# Autodesk Inventor assembly: WHEEL_BASE
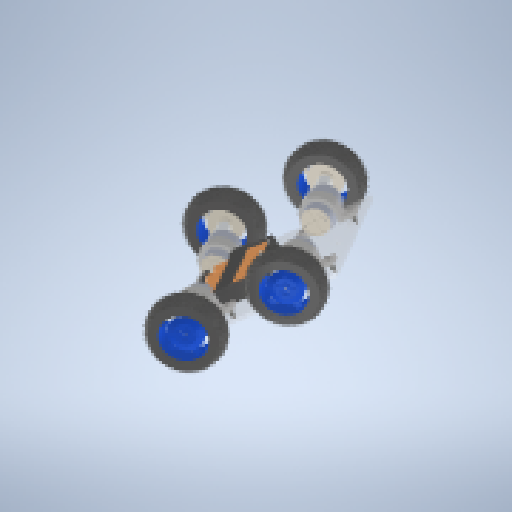
[picture p0: Inventor's stored thumbnail of the model, 512x512]
Saved by Autodesk Inventor 2025.3 (Build 293356030, 356C)
## iProperties
Created: 2026-06-30
Part Number: WHEEL_BASE
Document SubType Name: Assembly
Designer: user
Author: user
## Documents named in this file (6)
- C:\Docs\shcool\dojo\Design_3\Smaller\WHEEL_BASE.iam
- C:\Docs\shcool\dojo\Design_3\Smaller\base_2.ipt
- C:\Docs\shcool\dojo\Design_3\Smaller\motor_wheel_3.iam
- C:\Docs\shcool\dojo\Design_3\battery_case\Battery_Housing_Full.iam
- C:\Users\user\OneDrive\Documents\Inventor\Content Center Files\R2025\en-US\ISO 7040\DIEN EN ISO 7040 - M3.ipt
- C:\Users\user\OneDrive\Documents\Inventor\Content Center Files\R2025\en-US\ISO 4762(2)\ISO 4762 - M3 x 16ISO.ipt
## Components (22 placed, 5 different names)
1. base_2:1 — Mate:2, Mate:4, Mate:5, Mate:6, Mate:8, Mate:9, Mate:10, Mate:11, Mate:14, Mate:15, Mate:16, Mate:17, Mate:18, Insert:9, Insert:11, Insert:12, Insert:13, Insert:14, Insert:15, Insert:16, Insert:17
2. motor_wheel_3:1 [sub-assembly] — Mate:2, Mate:15, Mate:16, Insert:5, Insert:6
3. motor_wheel_3:2 [sub-assembly] — Mate:4, Mate:5, Mate:11, Insert:7, Insert:8
4. motor_wheel_3:3 [sub-assembly] — Mate:6, Mate:17, Mate:18, Insert:1, Insert:2
5. motor_wheel_3:4 [sub-assembly] — Mate:8, Mate:9, Mate:10, Mate:19, Insert:3, Insert:4
6. Battery_Housing_Full:1 [sub-assembly] — Mate:14, Mate:19
7. ISO 4762 M3 x 16:1 — Insert:5
8. ISO 4762 M3 x 16:2 — Insert:2
9. ISO 4762 M3 x 16:3 — Insert:3
10. ISO 4762 M3 x 16:4 — Insert:4
11. ISO 4762 M3 x 16:5 — Insert:6
12. ISO 4762 M3 x 16:6 — Insert:1
13. ISO 4762 M3 x 16:7 — Insert:7
14. ISO 4762 M3 x 16:8 — Insert:8
15. DIN EN ISO 7040 M3:3 — Insert:11
16. DIN EN ISO 7040 M3:4 — Insert:15
17. DIN EN ISO 7040 M3:5 — Insert:12
18. DIN EN ISO 7040 M3:6 — Insert:14
19. DIN EN ISO 7040 M3:7 — Insert:13
20. DIN EN ISO 7040 M3:8 — Insert:9
21. DIN EN ISO 7040 M3:9 — Insert:16
22. DIN EN ISO 7040 M3:10 — Insert:17
## Relationships (30: Insert 16, Mate 14)
- Mate:2: base_2:1 ↔ motor_wheel_3:1
- Mate:4: base_2:1 ↔ motor_wheel_3:2
- Mate:5: base_2:1 ↔ motor_wheel_3:2
- Mate:6: base_2:1 ↔ motor_wheel_3:3
- Mate:8: base_2:1 ↔ motor_wheel_3:4
- Mate:9: base_2:1 ↔ motor_wheel_3:4
- Mate:10: base_2:1 ↔ motor_wheel_3:4
- Mate:11: base_2:1 ↔ motor_wheel_3:2
- Mate:14: base_2:1 ↔ Battery_Housing_Full:1
- Mate:15: base_2:1 ↔ motor_wheel_3:1
- Mate:16: base_2:1 ↔ motor_wheel_3:1
- Mate:17: base_2:1 ↔ motor_wheel_3:3
- Mate:18: base_2:1 ↔ motor_wheel_3:3
- Mate:19 (3 mm): motor_wheel_3:4 ↔ Battery_Housing_Full:1
- Insert:1: motor_wheel_3:3 ↔ ISO 4762 M3 x 16:6
- Insert:2: motor_wheel_3:3 ↔ ISO 4762 M3 x 16:2
- Insert:3: motor_wheel_3:4 ↔ ISO 4762 M3 x 16:3
- Insert:4: motor_wheel_3:4 ↔ ISO 4762 M3 x 16:4
- Insert:5: motor_wheel_3:1 ↔ ISO 4762 M3 x 16:1
- Insert:6: motor_wheel_3:1 ↔ ISO 4762 M3 x 16:5
- Insert:7: motor_wheel_3:2 ↔ ISO 4762 M3 x 16:7
- Insert:8: motor_wheel_3:2 ↔ ISO 4762 M3 x 16:8
- Insert:9: base_2:1 ↔ DIN EN ISO 7040 M3:8
- Insert:11: base_2:1 ↔ DIN EN ISO 7040 M3:3
- Insert:12: base_2:1 ↔ DIN EN ISO 7040 M3:5
- Insert:13: base_2:1 ↔ DIN EN ISO 7040 M3:7
- Insert:14: base_2:1 ↔ DIN EN ISO 7040 M3:6
- Insert:15: base_2:1 ↔ DIN EN ISO 7040 M3:4
- Insert:16: base_2:1 ↔ DIN EN ISO 7040 M3:9
- Insert:17: base_2:1 ↔ DIN EN ISO 7040 M3:10
